# Autodesk Inventor assembly: 8 inch mecanum with toughbox (Bottom left)
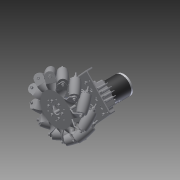
[picture p0: Inventor's stored thumbnail of the model, 180x180]
Saved by Autodesk Inventor 2014 (Build 180170000, 170)
## iProperties
Created: 2015-01-10
Part Number: 8 inch mecanum with toughbox (Bottom left)
Document SubType Name: Assembly
Designer: student
Author: student
## Documents named in this file (6)
- C:\Users\student\Documents\Inventor\2015 Recycle Rush\8 inch mecanum with toughbox (Bottom left).iam
- C:\Users\student\Documents\Inventor\Dillon And Justin\Derived Right Mecanum.ipt
- C:\Users\student\Documents\Inventor\2015 Recycle Rush\am-0077a-500 Key Hub r2.ipt
- C:\Users\student\Documents\Inventor\2015 Recycle Rush\Derived Toughbox mini.ipt
- C:\Users\student\Documents\Inventor\Dillon And Justin\Imported Components\MOT_CIM-Motor_217-2000.iam\MOT_CIM-Motor_217-2000.iam.iam
- MOT_CIM-Motor_217-2000.iam
## Components (4 placed, 4 different names)
1. Derived Right Mecanum:1 — Mate:1, Mate:2, Mate:3
2. am-0077a-500 Key Hub r2:2 — Mate:1, Mate:2, Mate:3, Mate:4, Mate:5
3. Derived Toughbox mini:1 — Mate:4, Mate:5, Mate:6, Mate:7
4. MOT_CIM-Motor_217-2000.iam:1 [sub-assembly] — Mate:6, Mate:7
## Relationships (7: Mate 7)
- Mate:1: Derived Right Mecanum:1 ↔ am-0077a-500 Key Hub r2:2
- Mate:2: Derived Right Mecanum:1 ↔ am-0077a-500 Key Hub r2:2
- Mate:3: Derived Right Mecanum:1 ↔ am-0077a-500 Key Hub r2:2
- Mate:4: am-0077a-500 Key Hub r2:2 ↔ Derived Toughbox mini:1
- Mate:5: am-0077a-500 Key Hub r2:2 ↔ Derived Toughbox mini:1
- Mate:6: Derived Toughbox mini:1 ↔ MOT_CIM-Motor_217-2000.iam:1
- Mate:7: Derived Toughbox mini:1 ↔ MOT_CIM-Motor_217-2000.iam:1
